# Autodesk Inventor assembly: Body V7 Pi5 - Removable Electronics
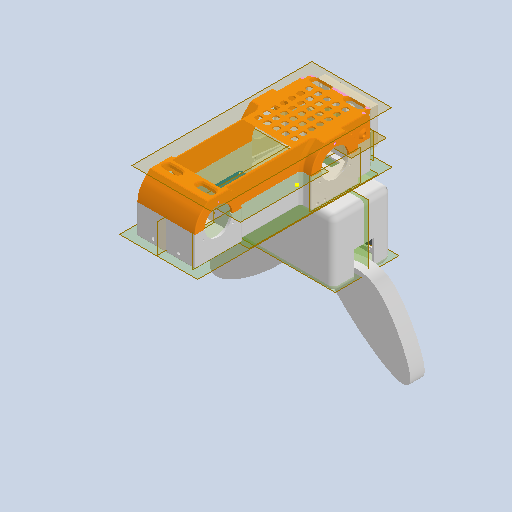
[picture p0: Inventor's stored thumbnail of the model, 512x512]
Saved by Autodesk Inventor 2024.2 (Build 282272000, 272)
## iProperties
Created: 2025-09-19
Part Number: Body V7 Pi5 - Removable Electronics
Document SubType Name: Assembly
Designer: AdminForWorker
Title: Body V7 Pi5 - Removable Electronics v36
Author: AdminForWorker
## Documents named in this file (15)
- D:\dog\construction\fox\body\тело лисы.iam
- D:\dog\construction\fox\boards\3D_PCB4_2024-01-15 v3.iam
- C:\dog\Pupper+v3\front_cable_clamp.ipt
- C:\dog\Pupper+v3\back_clamp.ipt
- C:\dog\Pupper+v3\Electronics tray - Integrated into body v38.iam
- C:\dog\Pupper+v3\ear - incut - springy - straight v5.iam
- D:\dog\construction\fox\legs\Part222.ipt
- D:\dog\construction\fox\body\верхняя часть.ipt
- D:\dog\construction\fox\body\крышка камера.ipt
- D:\dog\construction\fox\body\спина.ipt
- D:\dog\construction\fox\body\шея.ipt
- D:\dog\construction\fox\body\лицо.ipt
- D:\dog\construction\fox\body\голова потолок.ipt
- D:\dog\construction\fox\body\ухо правое.ipt
- D:\dog\construction\fox\raspberry\0329_экран.ipt
## Components (16 placed, 16 different names)
1. плата питания [sub-assembly] — Совмещение:3, Совмещение:4, Совмещение:5
2. крышка камера:1
3. переднее крепление правое
4. заднее крепление левое — Заподлицо:4, Заподлицо:5, Совмещение:1, Совмещение:2
5. заднее крепление правое — Заподлицо:4, Заподлицо:5, Совмещение:1
6. голова [sub-assembly]
7. переднее крепление левое
8. уши [sub-assembly]
9. основа тела — Заподлицо:1, Заподлицо:2, Заподлицо:3, Заподлицо:13
10. верхняя часть:1 — Заподлицо:1, Заподлицо:2, Заподлицо:3, Совмещение:2, Совмещение:3, Совмещение:4, Совмещение:5, Заподлицо:14, Заподлицо:16, Заподлицо:17, Заподлицо:18
11. потолок — Заподлицо:13, Заподлицо:14, Заподлицо:16, Заподлицо:17, Заподлицо:18, Заподлицо:19, Заподлицо:20
12. шея:1 — Заподлицо:19, Заподлицо:20
13. лицо:1 — Заподлицо:24, Заподлицо:25, Совмещение:6, Совмещение:7, Заподлицо:28
14. голова потолок:1 — Заподлицо:24, Заподлицо:25
15. ухо правое:1 — Заподлицо:26, Заподлицо:27
16. 0329_экран:1 — Совмещение:6, Совмещение:7, Заподлицо:28
## Relationships (29: Flush 22, Mate 7)
- Заподлицо:1 [Flush]: основа тела ↔ верхняя часть:1
- Заподлицо:2 [Flush]: основа тела ↔ верхняя часть:1
- Заподлицо:3 [Flush]: основа тела ↔ верхняя часть:1
- Заподлицо:4 [Flush]: заднее крепление левое ↔ заднее крепление правое
- Заподлицо:5 [Flush]: заднее крепление левое ↔ заднее крепление правое
- Совмещение:1 [Mate] (-30 mm): заднее крепление левое ↔ заднее крепление правое
- Совмещение:2 [Mate]: заднее крепление левое ↔ верхняя часть:1
- Совмещение:3 [Mate] (-15 mm): плата питания ↔ верхняя часть:1
- Совмещение:4 [Mate]: плата питания ↔ верхняя часть:1
- Совмещение:5 [Mate]: плата питания ↔ верхняя часть:1
- [Flush]: крышка камера:1 ↔ верхняя часть:1
- [Flush]: крышка камера:1 ↔ верхняя часть:1
- [Flush]: крышка камера:1 ↔ верхняя часть:1
- [Flush]: крышка камера:1 ↔ верхняя часть:1
- Заподлицо:13 [Flush]: основа тела ↔ потолок
- Заподлицо:14 [Flush]: верхняя часть:1 ↔ потолок
- Заподлицо:16 [Flush]: верхняя часть:1 ↔ потолок
- Заподлицо:17 [Flush]: верхняя часть:1 ↔ потолок
- Заподлицо:18 [Flush]: верхняя часть:1 ↔ потолок
- Заподлицо:19 [Flush]: потолок ↔ шея:1
- Заподлицо:20 [Flush]: потолок ↔ шея:1
- [Flush]: шея:1 ↔ лицо:1
- Заподлицо:24 [Flush]: лицо:1 ↔ голова потолок:1
- Заподлицо:25 [Flush]: лицо:1 ↔ голова потолок:1
- Заподлицо:26 [Flush]: ухо правое:1
- Заподлицо:27 [Flush]: ухо правое:1
- Совмещение:6 [Mate]: лицо:1 ↔ 0329_экран:1
- Совмещение:7 [Mate]: лицо:1 ↔ 0329_экран:1
- Заподлицо:28 [Flush]: лицо:1 ↔ 0329_экран:1
## Named parameters: d17_d6 = 0 mm
